# Autodesk Inventor assembly: Assembly1
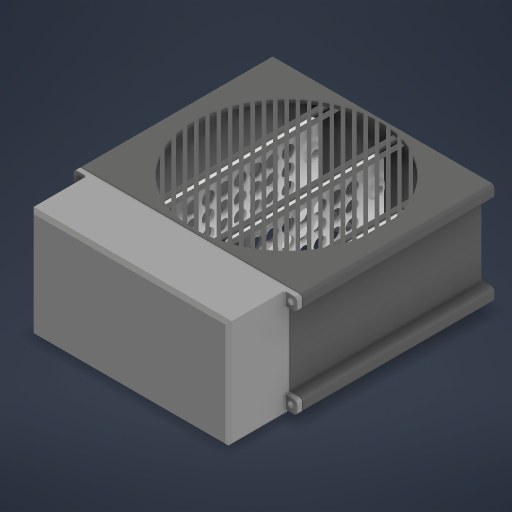
[picture p0: Inventor's stored thumbnail of the model, 512x512]
Saved by Autodesk Inventor 2024 (Build 280153000, 153)
## iProperties
Created: 2024-08-05
Part Number: Assembly1
Document SubType Name: Assembly
Designer: micjo
Author: micjo
## Documents named in this file (4)
- \\192.168.1.120\Main_4TB\mlandis\4TB_TN\Design_projects\Insight_Battery_Charger\v2\Assembly1.iam
- \\192.168.1.120\Main_4TB\mlandis\4TB_TN\Design_projects\Insight_Battery_Charger\v2\box.ipt
- \\192.168.1.120\Main_4TB\mlandis\4TB_TN\Design_projects\Insight_Battery_Charger\v2\lid.ipt
- \\192.168.1.120\Main_4TB\mlandis\4TB_TN\Design_projects\Insight_Battery_Charger\v2\drawer.ipt
## Components (5 placed, 3 different names)
1. box:1 — Mate:1, Mate:2, Mate:3, Mate:4, Mate:5, Mate:6, Mate:7
2. lid:1 — Mate:7
3. drawer:1 — Mate:1, Mate:2
4. drawer:2 — Mate:5, Mate:6
5. drawer:3 — Mate:3, Mate:4
## Relationships (7: Mate 7)
- Mate:1 (0.25 mm): box:1 ↔ drawer:1
- Mate:2 (0.2 mm): box:1 ↔ drawer:1
- Mate:3 (0.2 mm): box:1 ↔ drawer:3
- Mate:4 (0.2 mm): box:1 ↔ drawer:3
- Mate:5 (0.2 mm): box:1 ↔ drawer:2
- Mate:6 (0.2 mm): box:1 ↔ drawer:2
- Mate:7: box:1 ↔ lid:1
